# Autodesk Inventor assembly: 付け根ロール_1
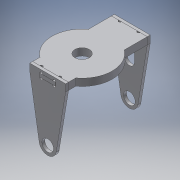
[picture p0: Inventor's stored thumbnail of the model, 180x180]
Saved by Autodesk Inventor 2018 (Build 220112000, 112)
## iProperties
Created: 2016-05-01
Part Number: 付け根ロール_1
Document SubType Name: Assembly
Designer: hiroaki
Mass: 95.2431 g
Surface Area: 199.324 cm^2
Volume: 15.6569 cm^3
Density: 6.08314 g/cm^3
Author: hiroaki
## Documents named in this file (4)
- Z:\OPR\OpenPlatform_ver1_0\下半身_160823\付け根ロール\付け根ロール_6.iam
- Z:\OPR\OpenPlatform_ver1_0\下半身_160823\付け根ロール\付け根ロール_メインフレーム_6_1.ipt
- Z:\OPR\OpenPlatform_ver1_0\下半身_160823\付け根ロール\付け根ロール_サブフレーム_6_5.ipt
- Z:\OPR\OpenPlatform_ver1_0\下半身_160823\付け根ロール\付け根ロール_サブフレーム_6_6.ipt
## Components (3 placed, 3 different names)
1. 付け根ロール_メインフレーム_6_1:1 — 挿入:52, 挿入:53, 挿入:54, 挿入:55
2. 付け根ロール_サブフレーム_6_5:1 — 挿入:52, 挿入:53
3. 付け根ロール_サブフレーム_6_6:1 — 挿入:54, 挿入:55
## Relationships (4: Insert 4)
- 挿入:52 [Insert]: 付け根ロール_メインフレーム_6_1:1 ↔ 付け根ロール_サブフレーム_6_5:1
- 挿入:53 [Insert]: 付け根ロール_メインフレーム_6_1:1 ↔ 付け根ロール_サブフレーム_6_5:1
- 挿入:54 [Insert]: 付け根ロール_メインフレーム_6_1:1 ↔ 付け根ロール_サブフレーム_6_6:1
- 挿入:55 [Insert]: 付け根ロール_メインフレーム_6_1:1 ↔ 付け根ロール_サブフレーム_6_6:1
